# Autodesk Inventor assembly: 知能ロボコン吸引部
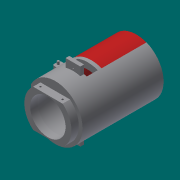
[picture p0: Inventor's stored thumbnail of the model, 180x180]
Saved by Autodesk Inventor 2013 (Build 170138000, 138)
## iProperties
Created: 2014-11-21
Part Number: 知能ロボコン吸引部
Document SubType Name: Assembly
Designer: horumo136
Author: horumo136
## Documents named in this file (4)
- C:\Users\horumo136\Documents\知能ロボコン吸引部.iam
- C:\Users\horumo136\Documents\知能ロボコン吸引部２.1.1.ipt
- C:\Users\horumo136\Documents\知能ロボコン吸引部２.1.2.ipt
- C:\Users\horumo136\Documents\3mmシャフト.ipt
## Components (3 placed, 3 different names)
1. 知能ロボコン吸引部２.1.1:1 — メイト:1
2. 知能ロボコン吸引部２.1.2:1 — メイト:2
3. 3mmシャフト:1 — メイト:1, メイト:2
## Relationships (2: Mate 2)
- メイト:1 [Mate]: 知能ロボコン吸引部２.1.1:1 ↔ 3mmシャフト:1
- メイト:2 [Mate]: 知能ロボコン吸引部２.1.2:1 ↔ 3mmシャフト:1
